# Autodesk Inventor assembly: Modul
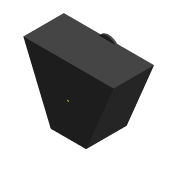
[picture p0: Inventor's stored thumbnail of the model, 180x180]
Saved by Autodesk Inventor 2018 (Build 220112000, 112)
## iProperties
Company: Fraunhofer ILT
Created: 2018-10-15
Part Number: Modul
Material: geeigneten Werkstoff auswählen !
Document SubType Name: Assembly
Designer: N.Grubert
Title: =Description
Author: N.Grubert
## Documents named in this file (6)
- C:\Users\knabe\Documents\Nicole\Uni\COSIMA\CAD\Detektormodul\Detektormodul.iam
- C:\Users\knabe\Documents\Nicole\Uni\COSIMA\CAD\Oktagongehäuse\Detektormodul Deckel.ipt
- C:\Users\knabe\Documents\Nicole\Uni\COSIMA\CAD\Oktagongehäuse\Detektormodul Gehäuse.ipt
- C:\Users\knabe\Documents\Nicole\Uni\COSIMA\CAD\Detektormodul\DetektorElektronik_Stage1.iam
- C:\Users\knabe\Documents\Nicole\Uni\COSIMA\CAD\Detektormodul\Stage2.ipt
- C:\Users\knabe\Documents\Nicole\Uni\COSIMA\CAD\Detektormodul\Photodiodendummie.ipt
## Components (8 placed, 5 different names)
1. Detektormodul Deckel:1 — Passend:1, Fluchtend:6, Fluchtend:7, Passend:8, Winkel:1, Fluchtend:8, Fluchtend:9, Passend:9, Passend:10, Passend:11
2. Detektormodul Gehäuse:1 — Passend:1, Passend:2, Passend:3, Passend:4, Fluchtend:6, Fluchtend:7, Passend:5, Passend:6, Passend:7, Passend:17
3. DetektorElektronik_Stage1:1 [sub-assembly] — Passend:5, Passend:6, Passend:7
4. Stage2:1 — Passend:8, Winkel:1, Fluchtend:8, Fluchtend:9, Passend:12, Passend:13, Passend:14, Passend:15, Passend:16, Passend:17
5. Photodiodendummie:1 — Passend:11, Passend:16
6. Photodiodendummie:2 — Passend:12, Passend:13
7. Photodiodendummie:3 — Passend:10, Passend:14
8. Photodiodendummie:4 — Passend:9, Passend:15
## Relationships (22: Mate 17, Flush 4, Angle 1)
- Passend:1 [Mate]: Detektormodul Deckel:1 ↔ Detektormodul Gehäuse:1
- Passend:2 [Mate]: Detektormodul Gehäuse:1
- Passend:3 [Mate]: Detektormodul Gehäuse:1
- Passend:4 [Mate]: Detektormodul Gehäuse:1
- Fluchtend:6 [Flush]: Detektormodul Deckel:1 ↔ Detektormodul Gehäuse:1
- Fluchtend:7 [Flush]: Detektormodul Deckel:1 ↔ Detektormodul Gehäuse:1
- Passend:5 [Mate]: Detektormodul Gehäuse:1 ↔ DetektorElektronik_Stage1:1
- Passend:6 [Mate] (0.5 mm): Detektormodul Gehäuse:1 ↔ DetektorElektronik_Stage1:1
- Passend:7 [Mate] (0.5 mm): Detektormodul Gehäuse:1 ↔ DetektorElektronik_Stage1:1
- Passend:8 [Mate]: Detektormodul Deckel:1 ↔ Stage2:1
- Winkel:1 [Angle] (0 deg): Detektormodul Deckel:1 ↔ Stage2:1
- Fluchtend:8 [Flush]: Detektormodul Deckel:1 ↔ Stage2:1
- Fluchtend:9 [Flush]: Detektormodul Deckel:1 ↔ Stage2:1
- Passend:9 [Mate]: Detektormodul Deckel:1 ↔ Photodiodendummie:4
- Passend:10 [Mate]: Detektormodul Deckel:1 ↔ Photodiodendummie:3
- Passend:11 [Mate]: Detektormodul Deckel:1 ↔ Photodiodendummie:1
- Passend:12 [Mate]: Stage2:1 ↔ Photodiodendummie:2
- Passend:13 [Mate]: Stage2:1 ↔ Photodiodendummie:2
- Passend:14 [Mate]: Stage2:1 ↔ Photodiodendummie:3
- Passend:15 [Mate]: Stage2:1 ↔ Photodiodendummie:4
- Passend:16 [Mate]: Stage2:1 ↔ Photodiodendummie:1
- Passend:17 [Mate]: Detektormodul Gehäuse:1 ↔ Stage2:1
